# Autodesk Inventor assembly: s-assy-link1
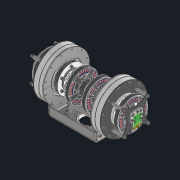
[picture p0: Inventor's stored thumbnail of the model, 180x180]
Saved by Autodesk Inventor 2021 (Build 250183000, 183)
## iProperties
Created: 2021-07-30
Part Number: s-assy-link1
Document SubType Name: Assembly
Designer: yuta0
Author: yuta0
## Documents named in this file (10)
- C:\Users\yuta0\Desktop\catchrobo_robot\s-assy-link1.iam
- C:\Users\yuta0\Desktop\catchrobo_robot\steel_plate6.ipt
- C:\Users\yuta0\Desktop\catchrobo_robot\s-assy-motor-wrist3.iam
- C:\Users\yuta0\Desktop\catchrobo_robot\s-assy-unit-j2.iam
- C:\Users\yuta0\Desktop\catchrobo_robot\s-assy-unit-j3.iam
- C:\Users\yuta0\Desktop\catchrobo_robot\steel_plate1.ipt
- C:\Users\yuta0\Desktop\catchrobo_robot\base9.ipt
- C:\Users\yuta0\Desktop\catchrobo_robot\steel_plate3.ipt
- C:\Users\yuta0\Desktop\catchrobo_robot\CB4-6.ipt
- C:\Users\yuta0\Desktop\catchrobo_robot\SFHRW8-75_7-M4-N4_s.ipt
## Components (26 placed, 9 different names)
1. steel_plate6:1 — メイト:7, メイト:8, メイト:9, メイト:10, メイト:11, メイト:12, メイト:13, メイト:14, メイト:15, メイト:16, メイト:17, メイト:18, メイト:23, メイト:28, メイト:29, メイト:30, メイト:38, メイト:39, メイト:40, メイト:41, メイト:42, メイト:43, メイト:44, メイト:49
2. s-assy-motor-wrist3:1 [sub-assembly] — メイト:13, メイト:15, メイト:17, メイト:54
3. s-assy-motor-wrist3:2 [sub-assembly] — メイト:14, メイト:16, メイト:18, メイト:34, メイト:35, メイト:36, メイト:37, メイト:45, メイト:46, メイト:47, メイト:48
4. s-assy-unit-j2:1 [sub-assembly] — メイト:7, メイト:8, メイト:9
5. s-assy-unit-j3:1 [sub-assembly] — メイト:10, メイト:11, メイト:12
6. steel_plate1:1 — メイト:23, メイト:28, メイト:50, メイト:51, メイト:52
7. steel_plate3:1 — メイト:29, メイト:30
8. base9:1 — メイト:38, メイト:39, メイト:40
9. CB4-6:6 — メイト:43, メイト:44
10. CB4-6:5 — メイト:41, メイト:42
11. CB4-6:9 — メイト:45, メイト:46
12. CB4-6:10 — メイト:47, メイト:48, メイト:53
13. CB4-6:1 — メイト:34, メイト:35
14. CB4-6:2 — メイト:36, メイト:37
15. CB4-6:13 — メイト:49, メイト:50
16. CB4-6:14 — メイト:51, メイト:52
17. SFHRW8-75_7-M4-N4_s:1 — メイト:53, メイト:54
18. CB4-6:7
19. CB4-6:8
20. CB4-6:11
21. CB4-6:12
22. CB4-6:15
23. CB4-6:16
24. CB4-6:17
25. CB4-6:18
26. SFHRW8-75_7-M4-N4_s:2
## Component patterns: (2 elements, first: CB4-6:6 + CB4-6:5 + CB4-6:9 + CB4-6:10 + CB4-6:1 + CB4-6:2 + CB4-6:13 + CB4-6:14 + SFHRW8-75_7-M4-N4_s:1)
## Relationships (37: Mate 37)
- メイト:7 [Mate]: steel_plate6:1 ↔ s-assy-unit-j2:1
- メイト:8 [Mate]: steel_plate6:1 ↔ s-assy-unit-j2:1
- メイト:9 [Mate]: steel_plate6:1 ↔ s-assy-unit-j2:1
- メイト:10 [Mate]: steel_plate6:1 ↔ s-assy-unit-j3:1
- メイト:11 [Mate]: steel_plate6:1 ↔ s-assy-unit-j3:1
- メイト:12 [Mate]: steel_plate6:1 ↔ s-assy-unit-j3:1
- メイト:13 [Mate]: steel_plate6:1 ↔ s-assy-motor-wrist3:1
- メイト:14 [Mate]: steel_plate6:1 ↔ s-assy-motor-wrist3:2
- メイト:15 [Mate]: steel_plate6:1 ↔ s-assy-motor-wrist3:1
- メイト:16 [Mate]: steel_plate6:1 ↔ s-assy-motor-wrist3:2
- メイト:17 [Mate]: steel_plate6:1 ↔ s-assy-motor-wrist3:1
- メイト:18 [Mate]: steel_plate6:1 ↔ s-assy-motor-wrist3:2
- メイト:23 [Mate]: steel_plate6:1 ↔ steel_plate1:1
- メイト:28 [Mate]: steel_plate6:1 ↔ steel_plate1:1
- メイト:29 [Mate]: steel_plate6:1 ↔ steel_plate3:1
- メイト:30 [Mate]: steel_plate6:1 ↔ steel_plate3:1
- メイト:34 [Mate]: s-assy-motor-wrist3:2 ↔ CB4-6:1
- メイト:35 [Mate]: s-assy-motor-wrist3:2 ↔ CB4-6:1
- メイト:36 [Mate]: s-assy-motor-wrist3:2 ↔ CB4-6:2
- メイト:37 [Mate]: s-assy-motor-wrist3:2 ↔ CB4-6:2
- メイト:38 [Mate]: steel_plate6:1 ↔ base9:1
- メイト:39 [Mate]: steel_plate6:1 ↔ base9:1
- メイト:40 [Mate]: steel_plate6:1 ↔ base9:1
- メイト:41 [Mate]: steel_plate6:1 ↔ CB4-6:5
- メイト:42 [Mate]: steel_plate6:1 ↔ CB4-6:5
- メイト:43 [Mate]: steel_plate6:1 ↔ CB4-6:6
- メイト:44 [Mate]: steel_plate6:1 ↔ CB4-6:6
- メイト:45 [Mate]: s-assy-motor-wrist3:2 ↔ CB4-6:9
- メイト:46 [Mate]: s-assy-motor-wrist3:2 ↔ CB4-6:9
- メイト:47 [Mate]: s-assy-motor-wrist3:2 ↔ CB4-6:10
- メイト:48 [Mate]: s-assy-motor-wrist3:2 ↔ CB4-6:10
- メイト:49 [Mate]: steel_plate6:1 ↔ CB4-6:13
- メイト:50 [Mate]: steel_plate1:1 ↔ CB4-6:13
- メイト:51 [Mate]: steel_plate1:1 ↔ CB4-6:14
- メイト:52 [Mate]: steel_plate1:1 ↔ CB4-6:14
- メイト:53 [Mate]: CB4-6:10 ↔ SFHRW8-75_7-M4-N4_s:1
- メイト:54 [Mate]: s-assy-motor-wrist3:1 ↔ SFHRW8-75_7-M4-N4_s:1
